# Autodesk Inventor assembly: Arm_Link_4
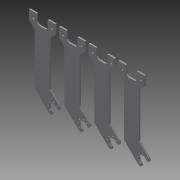
[picture p0: Inventor's stored thumbnail of the model, 180x180]
Saved by Autodesk Inventor 2013 (Build 170138000, 138)
## iProperties
Created: 2014-05-08
Part Number: Arm_Link_4
Document SubType Name: Assembly
Designer: andou
Author: andou
## Documents named in this file (2)
- C:\Users\andou\Documents\Inventor\RoboticsProject\project_4\Robot\CNC\Arm_Link_4.iam
- C:\Users\andou\Documents\Inventor\RoboticsProject\project_4\Robot\Arm\Arm_Link_yaw.ipt
## Components (4 placed, 1 different names)
1. Arm_Link_yaw:1
2. Arm_Link_yaw:2
3. Arm_Link_yaw:3
4. Arm_Link_yaw:4
## Component patterns: (4 elements, first: Arm_Link_yaw:1)
